# Autodesk Inventor assembly: Mecanismo Modelado
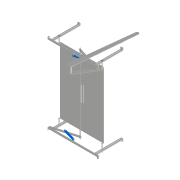
[picture p0: Inventor's stored thumbnail of the model, 180x180]
Saved by Autodesk Inventor 2021 (Build 250183000, 183)
## iProperties
Created: 2021-04-19
Part Number: Mecanismo Modelado
Document SubType Name: Assembly
Designer: carlo
Author: carlo
## Documents named in this file (12)
- C:\Users\carlo\Desktop\Concepto\Modelado Mecanismo\Mecanismo Modelado.iam
- C:\Users\carlo\Desktop\Concepto\Modelado Mecanismo\Bancada.ipt
- C:\Users\carlo\Desktop\Concepto\Modelado Mecanismo\Eslabon1.ipt
- C:\Users\carlo\Desktop\Concepto\Modelado Mecanismo\Eslabon2.ipt
- C:\Users\carlo\Desktop\Concepto\Modelado Mecanismo\Palanca.ipt
- C:\Users\carlo\Desktop\Concepto\Modelado Mecanismo\pin10.ipt
- C:\Users\carlo\Desktop\Concepto\Modelado Mecanismo\union.ipt
- C:\Users\carlo\Desktop\Concepto\Modelado Mecanismo\Bandeja.ipt
- C:\Users\carlo\Desktop\Concepto\Modelado Mecanismo\Pincerrado.ipt
- C:\Users\carlo\Desktop\Concepto\Modelado Mecanismo\PinCorto.ipt
- C:\Users\carlo\Desktop\Concepto\Modelado Mecanismo\PinLargo.ipt
- C:\Users\carlo\Desktop\Concepto\Modelado Mecanismo\arandela.ipt
## Components (22 placed, 11 different names)
1. Bancada:1 — Coincidencia:1, Nivelación:14, Nivelación:15, Coincidencia:7, Nivelación:16, Cilíndrica:24, Tangente:5
2. Eslabon1:1 — Coincidencia:1, Coincidencia:2, Cilíndrica:19, Coincidencia:9, Cilíndrica:23, Coincidencia:12
3. Eslabon2:1 — Coincidencia:2, Coincidencia:3, Cilíndrica:14, Nivelación:19, Cilíndrica:18, Coincidencia:8, Cilíndrica:25
4. Palanca:1 — Coincidencia:3, Coincidencia:4, Nivelación:5, Coincidencia:13
5. pin10:1 — Coincidencia:4, Nivelación:5
6. Bancada:2 — Nivelación:15, Coincidencia:7, Nivelación:16, Coincidencia:11, Cilíndrica:28, Tangente:6, Tangente:7, Tangente:8
7. Eslabon1:2 — Coincidencia:6, Cilíndrica:20, Coincidencia:11, Cilíndrica:27, Coincidencia:14
8. Eslabon2:2 — Coincidencia:6, Cilíndrica:15, Cilíndrica:21, Coincidencia:10, Cilíndrica:29, Coincidencia:15
9. union:1 — Cilíndrica:14, Cilíndrica:15, Cilíndrica:16, Nivelación:19, Coincidencia:17, Coincidencia:20, Coincidencia:24, Coincidencia:25
10. Bandeja:1 — Cilíndrica:16, Nivelación:14, Tangente:7, Tangente:8, Coincidencia:16, Coincidencia:18, Coincidencia:19, Coincidencia:21, Coincidencia:22, Coincidencia:23, Coincidencia:26, Coincidencia:27
11. Pincerrado:1 — Cilíndrica:18, Coincidencia:8, Cilíndrica:19, Coincidencia:9
12. Pincerrado:2 — Cilíndrica:20, Cilíndrica:21, Coincidencia:10
13. PinCorto:1 — Cilíndrica:23, Cilíndrica:24, Coincidencia:12
14. PinLargo:1 — Tangente:5, Cilíndrica:25, Coincidencia:13
15. PinCorto:2 — Cilíndrica:27, Cilíndrica:28, Coincidencia:14
16. Pincerrado:3 — Tangente:6, Cilíndrica:29, Coincidencia:15
17. arandela:1 — Coincidencia:16, Coincidencia:19
18. arandela:2 — Coincidencia:17, Coincidencia:20
19. arandela:3 — Coincidencia:18, Coincidencia:21
20. arandela:4 — Coincidencia:22, Coincidencia:23
21. arandela:5 — Coincidencia:24, Coincidencia:25
22. arandela:6 — Coincidencia:26, Coincidencia:27
## Relationships (48: Mate 26, CylindricalJoint 13, Flush 5, Tangent 4)
- Coincidencia:1 [Mate] (10 mm): Bancada:1 ↔ Eslabon1:1
- Coincidencia:2 [Mate] (3 mm): Eslabon1:1 ↔ Eslabon2:1
- Coincidencia:3 [Mate] (10 mm): Eslabon2:1 ↔ Palanca:1
- Coincidencia:4 [Mate]: Palanca:1 ↔ pin10:1
- Nivelación:5 [Flush]: Palanca:1 ↔ pin10:1
- Coincidencia:6 [Mate] (3 mm): Eslabon1:2 ↔ Eslabon2:2
- Cilíndrica:14 [CylindricalJoint]: Eslabon2:1 ↔ union:1
- Cilíndrica:15 [CylindricalJoint]: Eslabon2:2 ↔ union:1
- Cilíndrica:16 [CylindricalJoint]: union:1 ↔ Bandeja:1
- Nivelación:14 [Flush] (40 mm): Bancada:1 ↔ Bandeja:1
- Nivelación:15 [Flush]: Bancada:1 ↔ Bancada:2
- Coincidencia:7 [Mate] (-507.58 mm): Bancada:1 ↔ Bancada:2
- Nivelación:16 [Flush]: Bancada:1 ↔ Bancada:2
- Nivelación:19 [Flush] (-10 mm): Eslabon2:1 ↔ union:1
- Cilíndrica:18 [CylindricalJoint]: Eslabon2:1 ↔ Pincerrado:1
- Coincidencia:8 [Mate]: Eslabon2:1 ↔ Pincerrado:1
- Cilíndrica:19 [CylindricalJoint]: Eslabon1:1 ↔ Pincerrado:1
- Coincidencia:9 [Mate]: Eslabon1:1 ↔ Pincerrado:1
- Cilíndrica:20 [CylindricalJoint]: Eslabon1:2 ↔ Pincerrado:2
- Cilíndrica:21 [CylindricalJoint]: Eslabon2:2 ↔ Pincerrado:2
- Coincidencia:10 [Mate]: Eslabon2:2 ↔ Pincerrado:2
- Coincidencia:11 [Mate] (-20 mm): Bancada:2 ↔ Eslabon1:2
- Cilíndrica:23 [CylindricalJoint]: Eslabon1:1 ↔ PinCorto:1
- Cilíndrica:24 [CylindricalJoint]: Bancada:1 ↔ PinCorto:1
- Coincidencia:12 [Mate]: Eslabon1:1 ↔ PinCorto:1
- Tangente:5: Bancada:1 ↔ PinLargo:1
- Cilíndrica:25 [CylindricalJoint]: Eslabon2:1 ↔ PinLargo:1
- Coincidencia:13 [Mate]: Palanca:1 ↔ PinLargo:1
- Cilíndrica:27 [CylindricalJoint]: Eslabon1:2 ↔ PinCorto:2
- Cilíndrica:28 [CylindricalJoint]: Bancada:2 ↔ PinCorto:2
- Coincidencia:14 [Mate]: Eslabon1:2 ↔ PinCorto:2
- Tangente:6: Bancada:2 ↔ Pincerrado:3
- Cilíndrica:29 [CylindricalJoint]: Eslabon2:2 ↔ Pincerrado:3
- Coincidencia:15 [Mate]: Eslabon2:2 ↔ Pincerrado:3
- Tangente:7: Bancada:2 ↔ Bandeja:1
- Tangente:8: Bancada:2 ↔ Bandeja:1
- Coincidencia:16 [Mate]: Bandeja:1 ↔ arandela:1
- Coincidencia:17 [Mate]: union:1 ↔ arandela:2
- Coincidencia:18 [Mate]: Bandeja:1 ↔ arandela:3
- Coincidencia:19 [Mate]: Bandeja:1 ↔ arandela:1
- Coincidencia:20 [Mate]: union:1 ↔ arandela:2
- Coincidencia:21 [Mate]: Bandeja:1 ↔ arandela:3
- Coincidencia:22 [Mate]: Bandeja:1 ↔ arandela:4
- Coincidencia:23 [Mate]: Bandeja:1 ↔ arandela:4
- Coincidencia:24 [Mate]: union:1 ↔ arandela:5
- Coincidencia:25 [Mate]: union:1 ↔ arandela:5
- Coincidencia:26 [Mate]: Bandeja:1 ↔ arandela:6
- Coincidencia:27 [Mate]: Bandeja:1 ↔ arandela:6
